# Autodesk Inventor assembly: Printhead Assembly
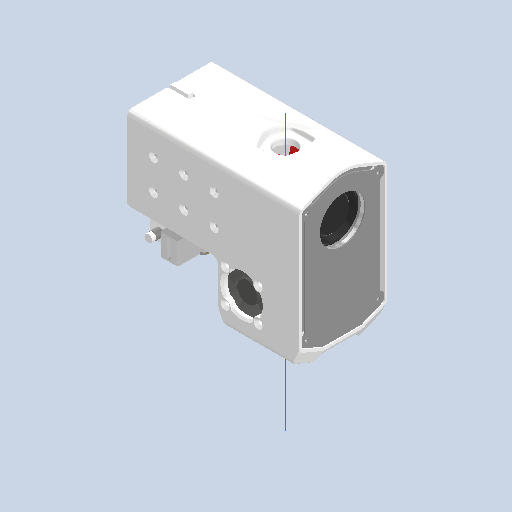
[picture p0: Inventor's stored thumbnail of the model, 512x512]
Saved by Autodesk Inventor 2024 (Build 280153000, 153)
## iProperties
Created: 2024-12-30
Part Number: Printhead Assembly
Document SubType Name: Assembly
Designer: Ishaan
Author: Ishaan
## Documents named in this file (17)
- E:\Projects\Axiom--IDEX-3D-Printer\CAD\05 - Printhead\Printhead Assembly.iam
- E:\Projects\Axiom--IDEX-3D-Printer\CAD\00 - COTS Components\MGN12H\MGN12H, LINEAR GUIDE BLOCK.ipt
- E:\Projects\Axiom--IDEX-3D-Printer\CAD\05 - Printhead\Printhead Baseplate.ipt
- E:\Projects\Axiom--IDEX-3D-Printer\CAD\00 - COTS Components\HGXLite Extruder\HGX-extruder\HGX-extruder.ipt
- E:\Projects\Axiom--IDEX-3D-Printer\CAD\00 - COTS Components\6mm Inductive Probe\6mm Inductive Probe.ipt
- E:\Projects\Axiom--IDEX-3D-Printer\CAD\00 - COTS Components\CHC Hotend\TD6S-CHC_mockup.iam
- E:\Projects\Axiom--IDEX-3D-Printer\CAD\05 - Printhead\Printhead Belt Retainer Cap.ipt
- E:\Projects\Axiom--IDEX-3D-Printer\CAD\05 - Printhead\Printhead Belt Retainer R2.ipt
- E:\Projects\Axiom--IDEX-3D-Printer\CAD\00 - COTS Components\3015 Fan\3015 Fan.ipt
- E:\Projects\Axiom--IDEX-3D-Printer\CAD\00 - COTS Components\Hardware\M3 25mm Standoff.ipt
- E:\Projects\Axiom--IDEX-3D-Printer\CAD\00 - COTS Components\Hardware\M3 10mm Standoff.ipt
- E:\Projects\Axiom--IDEX-3D-Printer\CAD\05 - Printhead\Hotend Cooling Fan Mount R2.ipt
- E:\Projects\Axiom--IDEX-3D-Printer\CAD\05 - Printhead\Printhead Cover Duct.ipt
- E:\Projects\Axiom--IDEX-3D-Printer\CAD\00 - COTS Components\5015 Fan\5015 Fan.ipt
- E:\Projects\Axiom--IDEX-3D-Printer\CAD\05 - Printhead\Printhead Endstop Cable Guide Plate.ipt
- E:\Projects\Axiom--IDEX-3D-Printer\CAD\00 - COTS Components\Hardware\SHCSM3x6.ipt
- E:\Projects\Axiom--IDEX-3D-Printer\CAD\00 - COTS Components\Hardware\SHCSM3x16.ipt
## Components (50 placed, 16 different names)
1. MGN12H, LINEAR GUIDE BLOCK:1 — Insert:23, Insert:24
2. Printhead Baseplate:1 — Insert:9, Insert:10, Insert:23, Insert:24, Insert:65, Insert:66, Angle:2, Insert:78, Insert:79, Insert:88, Insert:89, Insert:90, Insert:91, Insert:92, Insert:93, Insert:102, Insert:103, Insert:104, Insert:105, Insert:106, Insert:107, Insert:108, Insert:109
3. HGX-extruder:1 — Insert:9, Insert:10
4. 6mm Inductive Probe:1 — Mate:8, Flush:3
5. TD6S-CHC_mockup:1 [sub-assembly] — Mate:4, Insert:82, Insert:83
6. 3015 Fan:1 — Insert:86, Insert:87
7. Hotend Cooling Fan Mount R2:1 — Insert:78, Insert:79, Insert:82, Insert:83, Mate:7, Insert:86, Insert:87
8. Printhead Cover Duct:1 — Mate:6, Mate:7, Insert:84, Insert:85
9. 5015 Fan:1 — Insert:84, Insert:85
10. Printhead Endstop Cable Guide Plate:1 — Insert:94, Insert:95, Mate:8, Flush:3
11. SHCSM3x6:7 — Insert:105
12. SHCSM3x6:8 — Insert:104
13. SHCSM3x6:9 — Insert:103
14. SHCSM3x6:10 — Insert:102
15. SHCSM3x6:11 — Insert:109
16. SHCSM3x6:12 — Insert:107
17. SHCSM3x6:13 — Insert:106
18. SHCSM3x6:14 — Insert:108
19. SHCSM3x16:6 — Insert:115
20. SHCSM3x16:7 — Insert:116
21. SHCSM3x16:8 — Insert:117
22. SHCSM3x16:9 — Insert:118
23. SHCSM3x16:10 — Insert:119
24. Printhead Belt Retainer Cap:5 — Insert:119
25. Printhead Belt Retainer R2:5 — Insert:61, Insert:62, Insert:63, Insert:64
26. Printhead Belt Retainer Cap:6
27. Printhead Belt Retainer R2:6 — Insert:115, Insert:116, Insert:117, Insert:118
28. M3 10mm Standoff:1 — Insert:64, Insert:65
29. M3 10mm Standoff:2 — Insert:63
30. M3 10mm Standoff:3 — Insert:62
31. M3 10mm Standoff:4 — Insert:61, Insert:66
32. SHCSM3x16:1 — Insert:112
33. SHCSM3x16:2 — Insert:113
34. SHCSM3x16:3 — Insert:114
35. SHCSM3x16:4 — Insert:111
36. SHCSM3x16:5 — Insert:110
37. M3 25mm Standoff:1
38. M3 25mm Standoff:2 — Insert:51
39. M3 25mm Standoff:3
40. M3 25mm Standoff:4 — Insert:52
41. Printhead Belt Retainer Cap:3 — Insert:45, Insert:46
42. Printhead Belt Retainer R2:3 — Insert:45, Insert:46, Insert:51, Insert:52
43. Printhead Belt Retainer Cap:4 — Insert:49, Insert:50, Insert:110
44. Printhead Belt Retainer R2:4 — Insert:49, Insert:50, Insert:111, Insert:112, Insert:113, Insert:114
45. M3 25mm Standoff:5 — Insert:88, Insert:94
46. M3 25mm Standoff:6 — Insert:89
47. M3 25mm Standoff:7 — Insert:90, Insert:95
48. M3 25mm Standoff:8 — Insert:91
49. M3 25mm Standoff:9 — Insert:92
50. M3 25mm Standoff:10 — Insert:93
## Relationships (70: Insert 62, Mate 5, Flush 2, Angle 1)
- Insert:9: Printhead Baseplate:1 ↔ HGX-extruder:1
- Insert:10: Printhead Baseplate:1 ↔ HGX-extruder:1
- Insert:23: MGN12H, LINEAR GUIDE BLOCK:1 ↔ Printhead Baseplate:1
- Insert:24: MGN12H, LINEAR GUIDE BLOCK:1 ↔ Printhead Baseplate:1
- [Insert]: Printhead Baseplate:1 ↔ M3 25mm Standoff:4
- [Insert]: Printhead Baseplate:1 ↔ M3 25mm Standoff:3
- [Insert]: Printhead Baseplate:1 ↔ M3 25mm Standoff:2
- [Insert]: Printhead Baseplate:1 ↔ M3 25mm Standoff:1
- Insert:45: Printhead Belt Retainer Cap:3 ↔ Printhead Belt Retainer R2:3
- Insert:46: Printhead Belt Retainer Cap:3 ↔ Printhead Belt Retainer R2:3
- [Insert]: Printhead Belt Retainer R2:3 ↔ Printhead Belt Retainer R2:4
- [Insert]: Printhead Belt Retainer R2:3 ↔ Printhead Belt Retainer R2:4
- Insert:49: Printhead Belt Retainer Cap:4 ↔ Printhead Belt Retainer R2:4
- Insert:50: Printhead Belt Retainer Cap:4 ↔ Printhead Belt Retainer R2:4
- Insert:51: M3 25mm Standoff:2 ↔ Printhead Belt Retainer R2:3
- Insert:52: M3 25mm Standoff:4 ↔ Printhead Belt Retainer R2:3
- [Insert]: Printhead Belt Retainer Cap:5 ↔ Printhead Belt Retainer R2:5
- [Insert]: Printhead Belt Retainer Cap:5 ↔ Printhead Belt Retainer R2:5
- [Insert]: Printhead Belt Retainer R2:5 ↔ Printhead Belt Retainer R2:6
- [Insert]: Printhead Belt Retainer R2:5 ↔ Printhead Belt Retainer R2:6
- [Insert]: Printhead Belt Retainer Cap:6 ↔ Printhead Belt Retainer R2:6
- [Insert]: Printhead Belt Retainer Cap:6 ↔ Printhead Belt Retainer R2:6
- Insert:61: Printhead Belt Retainer R2:5 ↔ M3 10mm Standoff:4
- Insert:62: Printhead Belt Retainer R2:5 ↔ M3 10mm Standoff:3
- Insert:63: Printhead Belt Retainer R2:5 ↔ M3 10mm Standoff:2
- Insert:64: Printhead Belt Retainer R2:5 ↔ M3 10mm Standoff:1
- Insert:65: Printhead Baseplate:1 ↔ M3 10mm Standoff:1
- Insert:66: Printhead Baseplate:1 ↔ M3 10mm Standoff:4
- Mate:4: TD6S-CHC_mockup:1
- Mate:5
- Angle:2 (0 deg): Printhead Baseplate:1
- Flush:2 (-17 mm)
- Insert:78: Printhead Baseplate:1 ↔ Hotend Cooling Fan Mount R2:1
- Insert:79: Printhead Baseplate:1 ↔ Hotend Cooling Fan Mount R2:1
- Insert:82: TD6S-CHC_mockup:1 ↔ Hotend Cooling Fan Mount R2:1
- Insert:83: TD6S-CHC_mockup:1 ↔ Hotend Cooling Fan Mount R2:1
- Mate:6: Printhead Cover Duct:1
- Mate:7: Hotend Cooling Fan Mount R2:1 ↔ Printhead Cover Duct:1
- Insert:84: Printhead Cover Duct:1 ↔ 5015 Fan:1
- Insert:85: Printhead Cover Duct:1 ↔ 5015 Fan:1
- Insert:86: 3015 Fan:1 ↔ Hotend Cooling Fan Mount R2:1
- Insert:87: 3015 Fan:1 ↔ Hotend Cooling Fan Mount R2:1
- Insert:88: Printhead Baseplate:1 ↔ M3 25mm Standoff:5
- Insert:89: Printhead Baseplate:1 ↔ M3 25mm Standoff:6
- Insert:90: Printhead Baseplate:1 ↔ M3 25mm Standoff:7
- Insert:91: Printhead Baseplate:1 ↔ M3 25mm Standoff:8
- Insert:92: Printhead Baseplate:1 ↔ M3 25mm Standoff:9
- Insert:93: Printhead Baseplate:1 ↔ M3 25mm Standoff:10
- Insert:94: Printhead Endstop Cable Guide Plate:1 ↔ M3 25mm Standoff:5
- Insert:95: Printhead Endstop Cable Guide Plate:1 ↔ M3 25mm Standoff:7
- Mate:8: 6mm Inductive Probe:1 ↔ Printhead Endstop Cable Guide Plate:1
- Flush:3 (8 mm): 6mm Inductive Probe:1 ↔ Printhead Endstop Cable Guide Plate:1
- Insert:102: Printhead Baseplate:1 ↔ SHCSM3x6:10
- Insert:103: Printhead Baseplate:1 ↔ SHCSM3x6:9
- Insert:104: Printhead Baseplate:1 ↔ SHCSM3x6:8
- Insert:105: Printhead Baseplate:1 ↔ SHCSM3x6:7
- Insert:106: Printhead Baseplate:1 ↔ SHCSM3x6:13
- Insert:107: Printhead Baseplate:1 ↔ SHCSM3x6:12
- Insert:108: Printhead Baseplate:1 ↔ SHCSM3x6:14
- Insert:109: Printhead Baseplate:1 ↔ SHCSM3x6:11
- Insert:110: SHCSM3x16:5 ↔ Printhead Belt Retainer Cap:4
- Insert:111: SHCSM3x16:4 ↔ Printhead Belt Retainer R2:4
- Insert:112: SHCSM3x16:1 ↔ Printhead Belt Retainer R2:4
- Insert:113: SHCSM3x16:2 ↔ Printhead Belt Retainer R2:4
- Insert:114: SHCSM3x16:3 ↔ Printhead Belt Retainer R2:4
- Insert:115: SHCSM3x16:6 ↔ Printhead Belt Retainer R2:6
- Insert:116: SHCSM3x16:7 ↔ Printhead Belt Retainer R2:6
- Insert:117: SHCSM3x16:8 ↔ Printhead Belt Retainer R2:6
- Insert:118: SHCSM3x16:9 ↔ Printhead Belt Retainer R2:6
- Insert:119: SHCSM3x16:10 ↔ Printhead Belt Retainer Cap:5
## Named parameters: d45_d31 = 0 mm, d46_d32 = 0 mm, d47_d33 = 0 mm, d48_d34 = 0 mm, d49_d35 = 0 mm, d50_d36 = 0 mm, d55_d45_d31 = 0 mm, d56_d46_d32 = 0 mm, d57_d47_d33 = 0 mm, d58_d48_d34 = 0 mm, d59_d49_d35 = 0 mm, d60_d50_d36 = 0 mm
